# Autodesk Inventor assembly: motor_antigravity_4004_custom_shaft
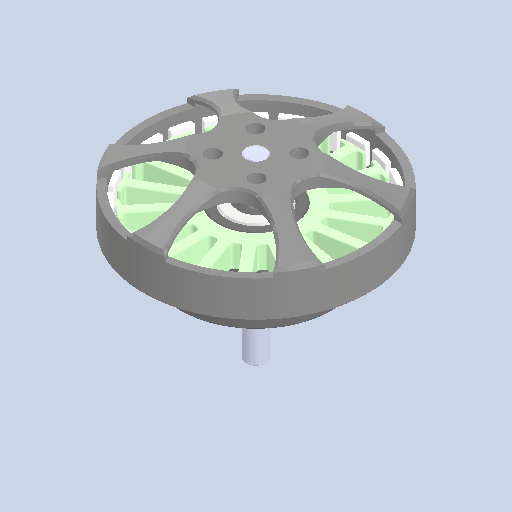
[picture p0: Inventor's stored thumbnail of the model, 512x512]
Saved by Autodesk Inventor 2023 (Build 270158000, 158)
## iProperties
Created: 2016-08-15
Part Number: motor_antigravity_4004_custom_shaft
Document SubType Name: Assembly
Designer: Jochen
Sending System: SolidWorks 2017
Last Author: Felix
Last Saved: 2020-06-08
Author: Jochen
## Documents named in this file (5)
- D:\Projects\Lisbeth\CAD\Tools\Motor Testbed\motor_antigravity_4004_custom_shaft.iam
- D:\Projects\Lisbeth\CAD\Tools\Motor Testbed\motor_antigravity_4004_stator.ipt
- D:\Projects\Lisbeth\CAD\Tools\Motor Testbed\motor_antigravity_4004_rotor.ipt
- D:\Projects\Lisbeth\CAD\Tools\Motor Testbed\motor_antigravity_4004_brass_spacer.ipt
- D:\Projects\Lisbeth\CAD\Common\Motor\Motor AntiGravity 4004  Custom Shaft.ipt
## Components (4 placed, 4 different names)
1. Motor AntiGravity 4004 Stator:1
2. Motor AntiGravity 4004 Rotor:1 — Mate:1, Mate:2
3. Motor AntiGravity 4004  Brass Spacer:1
4. Motor AntiGravity 4004 Custom Shaft — Mate:1, Mate:2
## Relationships (2: Mate 2)
- Mate:1: Motor AntiGravity 4004 Rotor:1 ↔ Motor AntiGravity 4004 Custom Shaft
- Mate:2: Motor AntiGravity 4004 Rotor:1 ↔ Motor AntiGravity 4004 Custom Shaft
